# Autodesk Inventor assembly: KelleWelle4.ipt
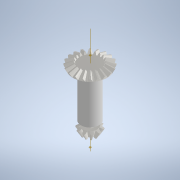
[picture p0: Inventor's stored thumbnail of the model, 180x180]
Saved by Autodesk Inventor 2021 (Build 250183000, 183)
## iProperties
Created: 2021-01-29
Part Number: KelleWelle4.ipt
Document SubType Name: Assembly
Designer: LETPJG
Author: LETPJG
## Documents named in this file (4)
- C:\Users\LETPJG\Documents\Vault\Gruppen\Gruppe 2\Entwurf\Amphibienfahrzeug\KelleWelle4.ipt.iam
- C:\Users\LETPJG\Documents\Vault\Gruppen\Gruppe 2\Entwurf\Amphibienfahrzeug\Planeten\Konstruktions-Assistent\Kegelrad12.ipt
- C:\Users\LETPJG\Documents\Vault\Gruppen\Gruppe 2\Entwurf\Amphibienfahrzeug\Planeten\Konstruktions-Assistent\Kegelrad22.ipt
- C:\Users\LETPJG\Documents\Vault\Gruppen\Gruppe 2\Entwurf\Amphibienfahrzeug\BauteilWelle4.ipt
## Components (3 placed, 3 different names)
1. Kegelrad1:1 — Einfügen:1
2. Kegelrad2:1 — Einfügen:2
3. BauteilWelle4:1 — Einfügen:1, Einfügen:2
## Relationships (2: Insert 2)
- Einfügen:1 [Insert]: Kegelrad1:1 ↔ BauteilWelle4:1
- Einfügen:2 [Insert]: Kegelrad2:1 ↔ BauteilWelle4:1
